# Autodesk Inventor assembly: шестерни прямые изменяемая траектория
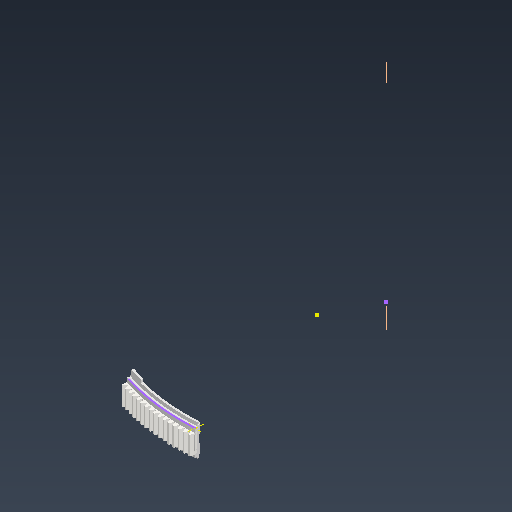
[picture p0: Inventor's stored thumbnail of the model, 512x512]
Saved by Autodesk Inventor 2026 (Build 300175000, 175)
## iProperties
Created: 2025-12-07
Part Number: шестерни прямые изменяемая траектория
Document SubType Name: Assembly
Designer: Phantom
Author: Phantom
## Documents named in this file (3)
- C:\Users\GameHD\Desktop\Phantom 16950\шестерни прямые изменяемая траектория.iam
- C:\Users\GameHD\Desktop\Phantom 16950\шестерни прямые изменяемая траектория\Мастер проектирования\Цилиндрическое зубчатое зацепление1.iam
- C:\Users\GameHD\Desktop\Phantom 16950\изменяемая траектория.ipt
## Components (2 placed, 2 different names)
1. Цилиндрическое зубчатое зацепление:1 [sub-assembly] — Совмещение:1, Заподлицо:4, Совмещение:3, Совмещение:4, Совмещение:5, Угол:1, Совмещение:6
2. изменяемая траектория:1 — Совмещение:1, Совмещение:2, Заподлицо:4, Совмещение:3, Совмещение:4, Угол:2, Совмещение:7
## Relationships (10: Mate 7, Angle 2, Flush 1)
- Совмещение:1 [Mate]: Цилиндрическое зубчатое зацепление:1 ↔ изменяемая траектория:1
- Совмещение:2 [Mate]: изменяемая траектория:1
- Заподлицо:4 [Flush] (10 mm): Цилиндрическое зубчатое зацепление:1 ↔ изменяемая траектория:1
- Совмещение:3 [Mate] (-10 mm): Цилиндрическое зубчатое зацепление:1 ↔ изменяемая траектория:1
- Совмещение:4 [Mate] (239 mm): Цилиндрическое зубчатое зацепление:1 ↔ изменяемая траектория:1
- Совмещение:5 [Mate]: Цилиндрическое зубчатое зацепление:1
- Угол:1 [Angle] (0 deg): Цилиндрическое зубчатое зацепление:1
- Совмещение:6 [Mate]: Цилиндрическое зубчатое зацепление:1
- Угол:2 [Angle] (0 deg): изменяемая траектория:1
- Совмещение:7 [Mate]: изменяемая траектория:1
